# Autodesk Inventor assembly: Tamale - V1p6p0
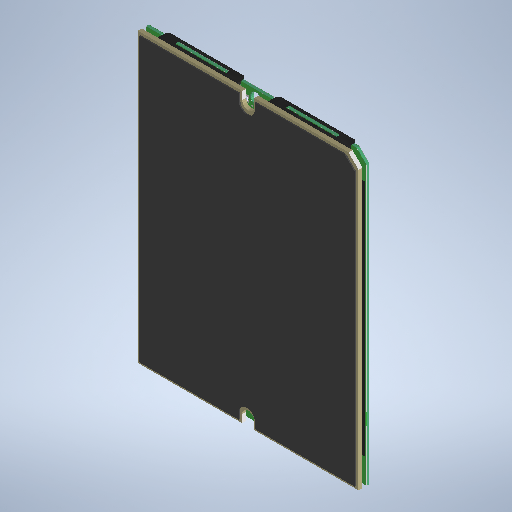
[picture p0: Inventor's stored thumbnail of the model, 512x512]
Saved by Autodesk Inventor 2025 (Build 290162000, 162)
## iProperties
Created: 2025-04-23
Part Number: Tamale - V1p6p0
Document SubType Name: Assembly
Designer: Caleb Fangmeier
Author: Caleb Fangmeier
## Documents named in this file (8)
- C:\Users\cfang\Desktop\nebraska-silicon-lab\Hardware\ETL\modules\Tamale v1.6\Tamale - V1p6p0.iam
- C:\Users\cfang\Desktop\nebraska-silicon-lab\Hardware\ETL\modules\Tamale v1.6\etl_etroc_module_v44\etl_etroc_module_v44.iam
- C:\Users\cfang\Desktop\nebraska-silicon-lab\Hardware\ETL\modules\Tamale v1.6\Sensor Placement Film.ipt
- C:\Users\cfang\Desktop\nebraska-silicon-lab\Hardware\ETL\modules\Tamale v1.6\BBM.iam
- C:\Users\cfang\Desktop\nebraska-silicon-lab\Hardware\ETL\modules\Tamale v1.6\Coverplate Film.ipt
- C:\Users\cfang\Desktop\nebraska-silicon-lab\Hardware\ETL\modules\Tamale v1.6\Baseplate v1.5.1.ipt
- C:\Users\cfang\Desktop\nebraska-silicon-lab\Hardware\ETL\modules\Tamale v1.6\Thermal Pad.ipt
- C:\Users\cfang\Desktop\nebraska-silicon-lab\Hardware\ETL\modules\Tamale v1.6\insert spacer - v4.ipt
## Components (13 placed, 7 different names)
1. etl_etroc_module_v44:1 [sub-assembly] — Mate:1, Angle:1, Flush:1, Flush:2, Angle:2, Angle:3, Angle:4, Angle:5, Flush:7, Flush:8, Angle:6, Flush:9, Flush:10, Angle:7, Flush:11, Flush:12, Angle:8, Angle:9, Angle:10, Angle:11, Mate:11, Mate:12, Mate:13, Mate:14, Mate:15, Mate:16, Mate:17, Mate:18, Mate:19, Mate:20, Mate:21, Mate:22
2. Sensor Placement Film:1 — Mate:1, Angle:1, Flush:1, Flush:2, Mate:2, Mate:3, Mate:4, Mate:5
3. BBM:1 [sub-assembly] — Mate:2, Angle:5, Mate:6, Flush:3, Flush:5
4. BBM:2 [sub-assembly] — Mate:3, Angle:4, Mate:6, Flush:3, Flush:4, Mate:7, Flush:7, Flush:8, Mate:8
5. BBM:3 [sub-assembly] — Mate:4, Angle:3, Flush:5, Flush:6
6. BBM:4 [sub-assembly] — Mate:5, Angle:2, Flush:4, Flush:6, Mate:7
7. Coverplate Film:1 — Mate:8, Angle:6, Flush:9, Flush:10, Mate:9
8. Baseplate v1.5.1:1 — Mate:9, Angle:7, Flush:11, Flush:12, Mate:10, Flush:13, Flush:14
9. Thermal Pad:1 — Mate:10, Flush:13, Flush:14
10. insert spacer - v4:1 — Angle:8, Mate:17, Mate:18, Mate:19
11. insert spacer - v4:2 — Angle:9, Mate:20, Mate:21, Mate:22
12. insert spacer - v4:3 — Angle:10, Mate:12, Mate:14, Mate:15
13. insert spacer - v4:4 — Angle:11, Mate:11, Mate:13, Mate:16
## Relationships (47: Mate 22, Flush 14, Angle 11)
- Mate:1: etl_etroc_module_v44:1 ↔ Sensor Placement Film:1
- Angle:1 (0 deg): etl_etroc_module_v44:1 ↔ Sensor Placement Film:1
- Flush:1 (0.25 mm): etl_etroc_module_v44:1 ↔ Sensor Placement Film:1
- Flush:2 (4.95 mm): etl_etroc_module_v44:1 ↔ Sensor Placement Film:1
- Mate:2: Sensor Placement Film:1 ↔ BBM:1
- Mate:3: Sensor Placement Film:1 ↔ BBM:2
- Mate:4: Sensor Placement Film:1 ↔ BBM:3
- Mate:5: Sensor Placement Film:1 ↔ BBM:4
- Angle:2 (0 deg): etl_etroc_module_v44:1 ↔ BBM:4
- Angle:3 (0 deg): etl_etroc_module_v44:1 ↔ BBM:3
- Angle:4 (0 deg): etl_etroc_module_v44:1 ↔ BBM:2
- Angle:5 (0 deg): etl_etroc_module_v44:1 ↔ BBM:1
- Mate:6 (0.2 mm): BBM:1 ↔ BBM:2
- Flush:3: BBM:1 ↔ BBM:2
- Flush:4: BBM:2 ↔ BBM:4
- Flush:5: BBM:1 ↔ BBM:3
- Flush:6: BBM:3 ↔ BBM:4
- Mate:7 (0.2 mm): BBM:2 ↔ BBM:4
- Flush:7 (0.55 mm): etl_etroc_module_v44:1 ↔ BBM:2
- Flush:8 (7.05 mm): etl_etroc_module_v44:1 ↔ BBM:2
- Mate:8: BBM:2 ↔ Coverplate Film:1
- Angle:6 (0 deg): etl_etroc_module_v44:1 ↔ Coverplate Film:1
- Flush:9 (1.05 mm): etl_etroc_module_v44:1 ↔ Coverplate Film:1
- Flush:10 (7.95 mm): etl_etroc_module_v44:1 ↔ Coverplate Film:1
- Mate:9: Coverplate Film:1 ↔ Baseplate v1.5.1:1
- Angle:7 (0 deg): etl_etroc_module_v44:1 ↔ Baseplate v1.5.1:1
- Flush:11: etl_etroc_module_v44:1 ↔ Baseplate v1.5.1:1
- Flush:12: etl_etroc_module_v44:1 ↔ Baseplate v1.5.1:1
- Mate:10: Baseplate v1.5.1:1 ↔ Thermal Pad:1
- Flush:13 (0.5 mm): Baseplate v1.5.1:1 ↔ Thermal Pad:1
- Flush:14 (0.5 mm): Baseplate v1.5.1:1 ↔ Thermal Pad:1
- Angle:8 (0 deg): etl_etroc_module_v44:1 ↔ insert spacer - v4:1
- Angle:9 (0 deg): etl_etroc_module_v44:1 ↔ insert spacer - v4:2
- Angle:10 (0 deg): etl_etroc_module_v44:1 ↔ insert spacer - v4:3
- Angle:11 (0 deg): etl_etroc_module_v44:1 ↔ insert spacer - v4:4
- Mate:11: etl_etroc_module_v44:1 ↔ insert spacer - v4:4
- Mate:12: etl_etroc_module_v44:1 ↔ insert spacer - v4:3
- Mate:13: etl_etroc_module_v44:1 ↔ insert spacer - v4:4
- Mate:14: etl_etroc_module_v44:1 ↔ insert spacer - v4:3
- Mate:15: etl_etroc_module_v44:1 ↔ insert spacer - v4:3
- Mate:16: etl_etroc_module_v44:1 ↔ insert spacer - v4:4
- Mate:17: etl_etroc_module_v44:1 ↔ insert spacer - v4:1
- Mate:18: etl_etroc_module_v44:1 ↔ insert spacer - v4:1
- Mate:19: etl_etroc_module_v44:1 ↔ insert spacer - v4:1
- Mate:20: etl_etroc_module_v44:1 ↔ insert spacer - v4:2
- Mate:21: etl_etroc_module_v44:1 ↔ insert spacer - v4:2
- Mate:22: etl_etroc_module_v44:1 ↔ insert spacer - v4:2
